# Autodesk Inventor assembly: GFRP_T2_02
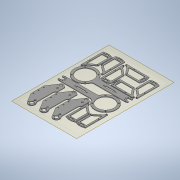
[picture p0: Inventor's stored thumbnail of the model, 180x180]
Saved by Autodesk Inventor 2020 (Build 240168000, 168)
## iProperties
Created: 2021-08-27
Part Number: GFRP_T2_02
Document SubType Name: Assembly
Designer: Masato
Author: Masato
## Documents named in this file (5)
- C:\Users\naoki\Documents\Inventor\CitBrains\git_clone\OpenPlatform4_1\GFRP_AT2_AT5_02\OpenPlatform_ver3_0\cam\GFRP_T2_02.iam
- C:\Users\naoki\Documents\Inventor\CitBrains\git_clone\OpenPlatform4_1\GFRP_AT2_AT5_02\OpenPlatform_ver3_0\cam\Disposable_Board.ipt
- C:\Users\naoki\Documents\Inventor\CitBrains\git_clone\OpenPlatform4_1\GFRP_AT2_AT5_02\OpenPlatform_ver3_0\LowerBody\Link\FrontLink_frame.ipt
- C:\Users\naoki\Documents\Inventor\CitBrains\git_clone\OpenPlatform4_1\GFRP_AT2_AT5_02\OpenPlatform_ver3_0\UpperBody\Arm\ForeArm_outside_frame.ipt
- C:\Users\naoki\Documents\Inventor\CitBrains\git_clone\OpenPlatform4_1\GFRP_AT2_AT5_02\OpenPlatform_ver3_0\UpperBody\Arm\UpperArm_side_frame.ipt
## Components (14 placed, 4 different names)
1. Disposable_Board:1 — メイト:2, メイト:1, フラッシュ:1, フラッシュ:2, メイト:4, フラッシュ:3, 正接:1, メイト:5, メイト:6, 角度:1, 角度:2, メイト:8, メイト:9, 角度:3, 正接:4, 正接:5, 角度:4, メイト:12, メイト:13, メイト:14, メイト:15, メイト:16, メイト:17, フラッシュ:5, フラッシュ:6, 角度:5
2. ForeArm_outside_frame:1 — メイト:8, 正接:2, 角度:3, 正接:3, 正接:5, 正接:6
3. ForeArm_outside_frame:2 — メイト:9, 正接:3, 正接:4, 角度:4, 正接:7, 正接:8, メイト:19, メイト:20
4. UpperArm_side_frame:1 — メイト:6, 角度:1, メイト:7, フラッシュ:4
5. UpperArm_side_frame:2 — メイト:5, 角度:2, メイト:7, メイト:10, 正接:2, フラッシュ:4
6. UpperArm_side_frame:3 — メイト:14, メイト:20, 正接:9, メイト:22
7. UpperArm_side_frame:4 — メイト:15, フラッシュ:5, 正接:7, メイト:18
8. UpperArm_side_frame:5 — メイト:13, 正接:8, メイト:18, メイト:21
9. UpperArm_side_frame:6 — メイト:12, メイト:19, 正接:10, メイト:21, メイト:22
10. UpperArm_side_frame:7 — メイト:16, 角度:5, 正接:10
11. UpperArm_side_frame:8 — メイト:17, 正接:9, フラッシュ:6
12. FrontLink_frame:1 — メイト:4, フラッシュ:3, 正接:1
13. FrontLink_frame:2
14. FrontLink_frame:3 — メイト:10, 正接:6
## Component patterns: (3 elements, first: FrontLink_frame:1)
## Relationships (41: Mate 20, Tangent 10, Flush 6, Angle 5)
- メイト:2 [Mate]: Disposable_Board:1
- メイト:1 [Mate]: Disposable_Board:1
- フラッシュ:1 [Flush]: Disposable_Board:1
- フラッシュ:2 [Flush]: Disposable_Board:1
- メイト:4 [Mate]: Disposable_Board:1 ↔ FrontLink_frame:1
- フラッシュ:3 [Flush] (2 mm): Disposable_Board:1 ↔ FrontLink_frame:1
- 正接:1 [Tangent] (2 mm): Disposable_Board:1 ↔ FrontLink_frame:1
- メイト:5 [Mate]: Disposable_Board:1 ↔ UpperArm_side_frame:2
- メイト:6 [Mate]: Disposable_Board:1 ↔ UpperArm_side_frame:1
- 角度:1 [Angle] (0 deg): Disposable_Board:1 ↔ UpperArm_side_frame:1
- 角度:2 [Angle] (0 deg): Disposable_Board:1 ↔ UpperArm_side_frame:2
- メイト:7 [Mate] (2.5 mm): UpperArm_side_frame:1 ↔ UpperArm_side_frame:2
- メイト:8 [Mate]: Disposable_Board:1 ↔ ForeArm_outside_frame:1
- メイト:9 [Mate]: Disposable_Board:1 ↔ ForeArm_outside_frame:2
- メイト:10 [Mate] (2.5 mm): UpperArm_side_frame:2 ↔ FrontLink_frame:3
- 正接:2 [Tangent] (2.5 mm): ForeArm_outside_frame:1 ↔ UpperArm_side_frame:2
- フラッシュ:4 [Flush]: UpperArm_side_frame:1 ↔ UpperArm_side_frame:2
- 角度:3 [Angle] (0 deg): Disposable_Board:1 ↔ ForeArm_outside_frame:1
- 正接:3 [Tangent] (2.5 mm): ForeArm_outside_frame:1 ↔ ForeArm_outside_frame:2
- 正接:4 [Tangent] (2.5 mm): Disposable_Board:1 ↔ ForeArm_outside_frame:2
- 正接:5 [Tangent] (4 mm): Disposable_Board:1 ↔ ForeArm_outside_frame:1
- 正接:6 [Tangent] (3 mm): ForeArm_outside_frame:1 ↔ FrontLink_frame:3
- 角度:4 [Angle] (0 deg): Disposable_Board:1 ↔ ForeArm_outside_frame:2
- メイト:12 [Mate]: Disposable_Board:1 ↔ UpperArm_side_frame:6
- メイト:13 [Mate]: Disposable_Board:1 ↔ UpperArm_side_frame:5
- メイト:14 [Mate]: Disposable_Board:1 ↔ UpperArm_side_frame:3
- メイト:15 [Mate]: Disposable_Board:1 ↔ UpperArm_side_frame:4
- メイト:16 [Mate]: Disposable_Board:1 ↔ UpperArm_side_frame:7
- メイト:17 [Mate]: Disposable_Board:1 ↔ UpperArm_side_frame:8
- フラッシュ:5 [Flush] (2 mm): Disposable_Board:1 ↔ UpperArm_side_frame:4
- 正接:7 [Tangent] (2.5 mm): ForeArm_outside_frame:2 ↔ UpperArm_side_frame:4
- 正接:8 [Tangent] (2.5 mm): ForeArm_outside_frame:2 ↔ UpperArm_side_frame:5
- メイト:18 [Mate] (2.5 mm): UpperArm_side_frame:4 ↔ UpperArm_side_frame:5
- メイト:19 [Mate] (2.5 mm): ForeArm_outside_frame:2 ↔ UpperArm_side_frame:6
- メイト:20 [Mate] (2.5 mm): ForeArm_outside_frame:2 ↔ UpperArm_side_frame:3
- 正接:9 [Tangent] (2.5 mm): UpperArm_side_frame:3 ↔ UpperArm_side_frame:8
- フラッシュ:6 [Flush] (4 mm): Disposable_Board:1 ↔ UpperArm_side_frame:8
- 角度:5 [Angle] (0 deg): Disposable_Board:1 ↔ UpperArm_side_frame:7
- 正接:10 [Tangent] (2.5 mm): UpperArm_side_frame:6 ↔ UpperArm_side_frame:7
- メイト:21 [Mate] (6 mm): UpperArm_side_frame:5 ↔ UpperArm_side_frame:6
- メイト:22 [Mate] (3 mm): UpperArm_side_frame:3 ↔ UpperArm_side_frame:6
